# Autodesk Inventor assembly: spiral assembly 1
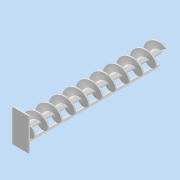
[picture p0: Inventor's stored thumbnail of the model, 180x180]
Saved by Autodesk Inventor 2020 (Build 240168000, 168)
## iProperties
Created: 2020-12-17
Part Number: spiral assembly 1
Document SubType Name: Assembly
Designer: solar
Author: solar
## Documents named in this file (4)
- D:\S.olar\College stuff\3 Junior\Term 5\MCT 131 Introductions to Mechatronics\FINAL INVENTOR\spiral assembly 1.iam
- D:\S.olar\College stuff\3 Junior\Term 5\MCT 131 Introductions to Mechatronics\FINAL INVENTOR\spiral base.ipt
- D:\S.olar\College stuff\3 Junior\Term 5\MCT 131 Introductions to Mechatronics\FINAL INVENTOR\spiral block.ipt
- D:\S.olar\College stuff\3 Junior\Term 5\MCT 131 Introductions to Mechatronics\FINAL INVENTOR\spiral shaft.ipt
## Components (3 placed, 3 different names)
1. spiral base:1 — Mate:1, Mate:2, Mate:3, Mate:5
2. spiral block:1 — Mate:1, Mate:2, Mate:3, Mate:4
3. spiral shaft:1 — Mate:4, Mate:5
## Relationships (5: Mate 5)
- Mate:1: spiral base:1 ↔ spiral block:1
- Mate:2: spiral base:1 ↔ spiral block:1
- Mate:3: spiral base:1 ↔ spiral block:1
- Mate:4: spiral block:1 ↔ spiral shaft:1
- Mate:5: spiral base:1 ↔ spiral shaft:1
